# Autodesk Inventor assembly: R2_ver1
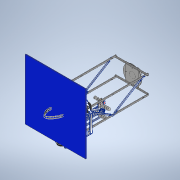
[picture p0: Inventor's stored thumbnail of the model, 180x180]
Saved by Autodesk Inventor 2021 (Build 250183000, 183)
## iProperties
Created: 2022-02-03
Part Number: R2_ver1
Document SubType Name: Assembly
Designer: hirohumi
Author: hirohumi
## Documents named in this file (12)
- C:\Users\hirohumi\OneDrive\ドキュメント\ロボ研\2022NHKロボコン\R2_version1\R2_ver1.iam
- C:\Users\hirohumi\OneDrive\ドキュメント\ロボ研\2022NHKロボコン\R2_version1\R2_オムニ.iam
- C:\Users\hirohumi\OneDrive\ドキュメント\ロボ研\2022NHKロボコン\フィールドCAD\スタートゾーン_blue area R1.ipt
- C:\Users\hirohumi\OneDrive\ドキュメント\ロボ研\2022NHKロボコン\R2_version1\R2_アーム部.iam
- C:\Users\hirohumi\OneDrive\ドキュメント\ロボ研\2022NHKロボコン\フィールドCAD\ボールオンヘッドを乗せる台.ipt
- C:\Users\hirohumi\OneDrive\ドキュメント\ロボ研\2022NHKロボコン\R2_version1\プレート保持_角柱1.ipt
- C:\Users\hirohumi\OneDrive\ドキュメント\ロボ研\2022NHKロボコン\R2_version1\プレート保持_固定具1.ipt
- C:\Users\hirohumi\OneDrive\ドキュメント\ロボ研\2022NHKロボコン\R2_version1\プレート保持_角柱2.ipt
- C:\Users\hirohumi\OneDrive\ドキュメント\ロボ研\2022NHKロボコン\R2_version1\プレート保持_角柱3.ipt
- C:\Users\hirohumi\OneDrive\ドキュメント\ロボ研\2022NHKロボコン\R2_version1\プレート保持_固定具3.ipt
- C:\Users\hirohumi\OneDrive\ドキュメント\ロボ研\2022NHKロボコン\R2_version1\プレート保持_固定具2.ipt
- C:\Users\hirohumi\OneDrive\ドキュメント\ロボ研\2022NHKロボコン\R2_version1\プレート保持_いた.ipt
## Components (25 placed, 11 different names)
1. R2_オムニ:1 [sub-assembly] — 正接:1, 正接:2, 正接:3, 挿入:1, 挿入:2, 挿入:3, 挿入:4, 挿入:5, 挿入:6, 挿入:7, 挿入:8, 挿入:9, 挿入:10
2. スタートゾーン_blue area R1:1 — 正接:1, 正接:2, 正接:3
3. R2_アーム部:1 [sub-assembly] — 挿入:1, 挿入:2
4. ボールオンヘッドを乗せる台:1 — 挿入:44, 挿入:45
5. プレート保持_角柱1:1 — 挿入:15, 挿入:16, 挿入:20, 挿入:22, 挿入:23, 挿入:26, 挿入:27
6. プレート保持_角柱1:2 — 挿入:17, 挿入:18, 挿入:19, 挿入:30, 挿入:31
7. プレート保持_角柱1:3 — 挿入:13, 挿入:14, 挿入:32, 挿入:33
8. プレート保持_角柱1:4 — 挿入:11, 挿入:12, 挿入:21, 挿入:24, 挿入:25, 挿入:28, 挿入:29
9. プレート保持_固定具1:1 — 挿入:3, 挿入:4, 挿入:15, 挿入:16
10. プレート保持_固定具1:2 — 挿入:5, 挿入:6, 挿入:17, 挿入:18
11. プレート保持_固定具1:3 — 挿入:7, 挿入:8, 挿入:11, 挿入:12
12. プレート保持_固定具1:4 — 挿入:9, 挿入:10, 挿入:13, 挿入:14
13. プレート保持_角柱2:1 — 挿入:19
14. プレート保持_角柱2:2 — 挿入:20, 挿入:21, 挿入:42, 挿入:43
15. プレート保持_角柱3:1 — 挿入:40, 挿入:41
16. プレート保持_角柱3:2 — 挿入:38, 挿入:39
17. プレート保持_角柱3:3 — 挿入:36, 挿入:37
18. プレート保持_角柱3:4 — 挿入:34, 挿入:35
19. プレート保持_固定具3:1 — 挿入:24, 挿入:25, 挿入:38
20. プレート保持_固定具3:2 — 挿入:28, 挿入:29, 挿入:40
21. プレート保持_固定具2:1 — 挿入:30, 挿入:31, 挿入:35, 挿入:36
22. プレート保持_固定具2:2 — 挿入:32, 挿入:33, 挿入:39, 挿入:41
23. プレート保持_固定具3:3 — 挿入:26, 挿入:27, 挿入:37
24. プレート保持_固定具3:4 — 挿入:22, 挿入:23, 挿入:34
25. プレート保持_いた:1 — 挿入:42, 挿入:43, 挿入:44, 挿入:45
## Relationships (48: Insert 45, Tangent 3)
- 正接:1 [Tangent]: R2_オムニ:1 ↔ スタートゾーン_blue area R1:1
- 正接:2 [Tangent]: R2_オムニ:1 ↔ スタートゾーン_blue area R1:1
- 正接:3 [Tangent]: R2_オムニ:1 ↔ スタートゾーン_blue area R1:1
- 挿入:1 [Insert]: R2_オムニ:1 ↔ R2_アーム部:1
- 挿入:2 [Insert]: R2_オムニ:1 ↔ R2_アーム部:1
- 挿入:3 [Insert]: R2_オムニ:1 ↔ プレート保持_固定具1:1
- 挿入:4 [Insert]: R2_オムニ:1 ↔ プレート保持_固定具1:1
- 挿入:5 [Insert]: R2_オムニ:1 ↔ プレート保持_固定具1:2
- 挿入:6 [Insert]: R2_オムニ:1 ↔ プレート保持_固定具1:2
- 挿入:7 [Insert]: R2_オムニ:1 ↔ プレート保持_固定具1:3
- 挿入:8 [Insert]: R2_オムニ:1 ↔ プレート保持_固定具1:3
- 挿入:9 [Insert]: R2_オムニ:1 ↔ プレート保持_固定具1:4
- 挿入:10 [Insert]: R2_オムニ:1 ↔ プレート保持_固定具1:4
- 挿入:11 [Insert]: プレート保持_角柱1:4 ↔ プレート保持_固定具1:3
- 挿入:12 [Insert]: プレート保持_角柱1:4 ↔ プレート保持_固定具1:3
- 挿入:13 [Insert]: プレート保持_角柱1:3 ↔ プレート保持_固定具1:4
- 挿入:14 [Insert]: プレート保持_角柱1:3 ↔ プレート保持_固定具1:4
- 挿入:15 [Insert]: プレート保持_角柱1:1 ↔ プレート保持_固定具1:1
- 挿入:16 [Insert]: プレート保持_角柱1:1 ↔ プレート保持_固定具1:1
- 挿入:17 [Insert]: プレート保持_角柱1:2 ↔ プレート保持_固定具1:2
- 挿入:18 [Insert]: プレート保持_角柱1:2 ↔ プレート保持_固定具1:2
- 挿入:19 [Insert]: プレート保持_角柱1:2 ↔ プレート保持_角柱2:1
- 挿入:20 [Insert]: プレート保持_角柱1:1 ↔ プレート保持_角柱2:2
- 挿入:21 [Insert]: プレート保持_角柱1:4 ↔ プレート保持_角柱2:2
- 挿入:22 [Insert]: プレート保持_角柱1:1 ↔ プレート保持_固定具3:4
- 挿入:23 [Insert]: プレート保持_角柱1:1 ↔ プレート保持_固定具3:4
- 挿入:24 [Insert]: プレート保持_角柱1:4 ↔ プレート保持_固定具3:1
- 挿入:25 [Insert]: プレート保持_角柱1:4 ↔ プレート保持_固定具3:1
- 挿入:26 [Insert]: プレート保持_角柱1:1 ↔ プレート保持_固定具3:3
- 挿入:27 [Insert]: プレート保持_角柱1:1 ↔ プレート保持_固定具3:3
- 挿入:28 [Insert]: プレート保持_角柱1:4 ↔ プレート保持_固定具3:2
- 挿入:29 [Insert]: プレート保持_角柱1:4 ↔ プレート保持_固定具3:2
- 挿入:30 [Insert]: プレート保持_角柱1:2 ↔ プレート保持_固定具2:1
- 挿入:31 [Insert]: プレート保持_角柱1:2 ↔ プレート保持_固定具2:1
- 挿入:32 [Insert]: プレート保持_角柱1:3 ↔ プレート保持_固定具2:2
- 挿入:33 [Insert]: プレート保持_角柱1:3 ↔ プレート保持_固定具2:2
- 挿入:34 [Insert]: プレート保持_角柱3:4 ↔ プレート保持_固定具3:4
- 挿入:35 [Insert]: プレート保持_角柱3:4 ↔ プレート保持_固定具2:1
- 挿入:36 [Insert]: プレート保持_角柱3:3 ↔ プレート保持_固定具2:1
- 挿入:37 [Insert]: プレート保持_角柱3:3 ↔ プレート保持_固定具3:3
- 挿入:38 [Insert]: プレート保持_角柱3:2 ↔ プレート保持_固定具3:1
- 挿入:39 [Insert]: プレート保持_角柱3:2 ↔ プレート保持_固定具2:2
- 挿入:40 [Insert]: プレート保持_角柱3:1 ↔ プレート保持_固定具3:2
- 挿入:41 [Insert]: プレート保持_角柱3:1 ↔ プレート保持_固定具2:2
- 挿入:42 [Insert]: プレート保持_角柱2:2 ↔ プレート保持_いた:1
- 挿入:43 [Insert]: プレート保持_角柱2:2 ↔ プレート保持_いた:1
- 挿入:44 [Insert]: ボールオンヘッドを乗せる台:1 ↔ プレート保持_いた:1
- 挿入:45 [Insert]: ボールオンヘッドを乗せる台:1 ↔ プレート保持_いた:1
